# Autodesk Inventor assembly: Structure
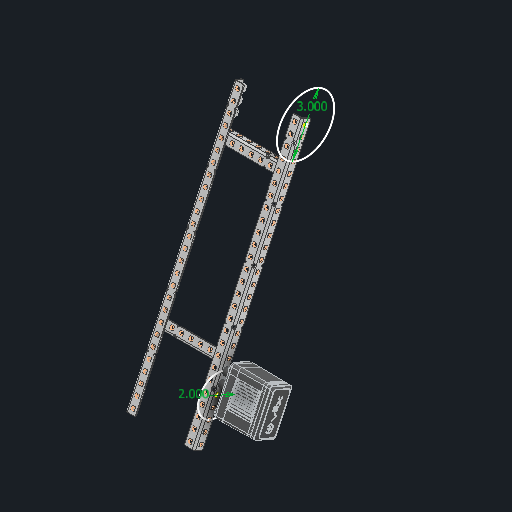
[picture p0: Inventor's stored thumbnail of the model, 512x512]
Saved by Autodesk Inventor 2025 (Build 290162000, 162)
## iProperties
Created: 2024-12-25
Part Number: Structure
Document SubType Name: Assembly
Designer: Averey Ku
Author: Averey Ku
## Documents named in this file (6)
- D:\VEX\High Stakes\CAD\V4\Conveyer\Structure.iam
- D:\VEX\High Stakes\CAD\ROBOPROS-CAD-Inventor\Structure\Angle\Aluminum 1x1\Alu Angle 1x1x27.ipt
- D:\VEX\High Stakes\CAD\ROBOPROS-CAD-Inventor\Electronics\Motors with Screws\SteelM-StarS.iam
- D:\VEX\High Stakes\CAD\ROBOPROS-CAD-Inventor\Electronics\Motors with Screws.iam
- D:\VEX\High Stakes\CAD\ROBOPROS-CAD-Inventor\Structure\Angle\Aluminum 1x1\Alu Angle 1x1x7.ipt
- D:\VEX\High Stakes\CAD\ROBOPROS-CAD-Inventor\Motion\Shaft LS\Bearing Flat Low Profile.ipt
## Components (7 placed, 4 different names)
1. Alu Angle 1x1x27:1 — Insert:2, Mate:2, Insert:4, Insert:5
2. SteelM-StarS:1 [sub-assembly]
3. Alu Angle 1x1x27:2 — Insert:3, Mate:3, Insert:6, Mate:5
4. Alu Angle 1x1x7:1 — Insert:4, Mate:4, Insert:6
5. Alu Angle 1x1x7:2 — Insert:5, Mate:4, Mate:5
6. Bearing Flat Low Profile:1 — Insert:2, Mate:2
7. Bearing Flat Low Profile:2 — Insert:3, Mate:3
## Relationships (11: Insert 6, Mate 5)
- [Insert]: Alu Angle 1x1x27:1 ↔ SteelM-StarS:1
- [Mate]: Alu Angle 1x1x27:1 ↔ SteelM-StarS:1
- Insert:2: Alu Angle 1x1x27:1 ↔ Bearing Flat Low Profile:1
- Mate:2: Alu Angle 1x1x27:1 ↔ Bearing Flat Low Profile:1
- Insert:3: Alu Angle 1x1x27:2 ↔ Bearing Flat Low Profile:2
- Mate:3: Alu Angle 1x1x27:2 ↔ Bearing Flat Low Profile:2
- Insert:4: Alu Angle 1x1x27:1 ↔ Alu Angle 1x1x7:1
- Insert:5: Alu Angle 1x1x27:1 ↔ Alu Angle 1x1x7:2
- Mate:4: Alu Angle 1x1x7:1 ↔ Alu Angle 1x1x7:2
- Insert:6: Alu Angle 1x1x27:2 ↔ Alu Angle 1x1x7:1
- Mate:5: Alu Angle 1x1x27:2 ↔ Alu Angle 1x1x7:2
